# Autodesk Inventor assembly: 100-02
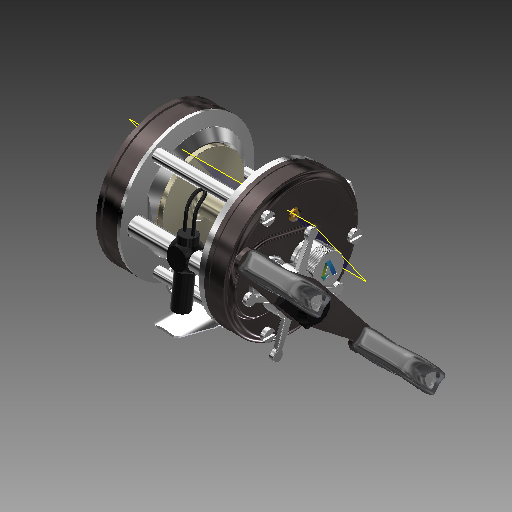
[picture p0: Inventor's stored thumbnail of the model, 512x512]
Saved by Autodesk Inventor 2019 (Build 230136000, 136)
## iProperties
Company: Autodesk Inc.
Created: 2017-06-27
Part Number: 100-02
Document SubType Name: Assembly
Designer: Autodesk Inc.
Mass: 263.654 g
Surface Area: 969.622 cm^2
Volume: 67.9846 cm^3
Density: 3.87815 g/cm^3
Author: Inventor
## Documents named in this file (31)
- C:\TEMP\Fishing Rod\Workspaces\_Fishing Reel Assembly.iam
- C:\TEMP\Fishing Rod\Workspaces\Reel Cage Assembly.iam
- C:\TEMP\Fishing Rod\Workspaces\Spool Assembly.iam
- C:\TEMP\Fishing Rod\Workspaces\Winding Assembly.iam
- C:\TEMP\Fishing Rod\Workspaces\Crankshaft Assembly.iam
- C:\TEMP\Fishing Rod\Workspaces\Crankshaft Spacer Tension Spring.ipt
- C:\TEMP\Fishing Rod\Workspaces\Handle Side Cover Assembly.iam
- C:\TEMP\Fishing Rod\Workspaces\Captive Cover Screw.ipt
- C:\TEMP\Fishing Rod\Workspaces\Plastic Bushing.ipt
- C:\TEMP\Fishing Rod\Workspaces\Front Drive Transfer Gear.iam
- C:\TEMP\Fishing Rod\Workspaces\Drag Adjustment Handle.ipt
- C:\TEMP\Fishing Rod\Workspaces\Plastic Crankshaft Spacer.ipt
- C:\TEMP\Fishing Rod\Workspaces\Spring Spacer.ipt
- C:\TEMP\Fishing Rod\Workspaces\Winding Handle.iam
- C:\TEMP\Fishing Rod\Workspaces\Crankshaft Cover.ipt
- C:\TEMP\Fishing Rod\Workspaces\Line Guide Tail Busing.ipt
- C:\TEMP\Fishing Rod\Workspaces\Line Guide Drive Shaft.ipt
- C:\TEMP\Fishing Rod\Workspaces\Follower Guide Pin Retainer.ipt
- C:\TEMP\Fishing Rod\Workspaces\Follower Guide Pin.ipt
- C:\TEMP\Fishing Rod\Workspaces\Line Guide.ipt
- C:\TEMP\Fishing Rod\Workspaces\Line Guide Shaft Housing.ipt
- C:\TEMP\Fishing Rod\Workspaces\Line Guide Head Bushing.ipt
- C:\TEMP\Fishing Rod\Workspaces\Locking Plate.ipt
- C:\TEMP\Fishing Rod\Workspaces\Winder Transfer Gear Spindle.ipt
- C:\TEMP\Fishing Rod\Workspaces\Winder Transfer Gear.iam
- C:\TEMP\Fishing Rod\Workspaces\Back Side Cover Assembly.iam
- C:\TEMP\Fishing Rod\Workspaces\Front Drive Transfer Gear\Design Accelerator\Bearing1.iam
- C:\TEMP\Fishing Rod\Workspaces\Main Bearing Cover.ipt
- C:\TEMP\Fishing Rod\Libraries\Content Center Files\en-US\ANSI B18.6.7M(03)\ANSI B18.6.7M - M2x0.4 x 6(3).ipt
- C:\TEMP\Fishing Rod\Libraries\Content Center Files\en-US\BS 4183(5)\BS 4183 - M3 x 5(2) I.ipt
- C:\TEMP\Fishing Rod\Workspaces\Back Drive Transfer Gear.iam
## Components (37 placed, 30 different names)
1. Reel Cage Assembly:1 [sub-assembly] — Mate:1, Insert:1, Mate:2, Angle:7, Insert:15, Mate:23, Mate:26, Mate:27, Mate:35, Mate:36, Tangent:6
2. Spool Assembly:1 [sub-assembly] — Mate:1, Mate:6, Mate:7, Tangent:2, Mate:8, Rotation:2, Rotation:3, Mate:20, Flush:1, Mate:27, Mate:34
3. Winding Assembly:1 [sub-assembly] — Insert:1, Mate:2, Insert:2, Insert:3, Mate:11
4. Crankshaft Assembly:1 [sub-assembly] — Insert:2, Mate:3, Angle:1, Mate:4, Angle:2, Mate:10, Angle:3, Angle:4, Rotation:1, Mate:29, Mate:30, Mate:37, Rotation:7
5. Crankshaft Spacer Tension Spring:1 — Mate:3, Angle:1, Mate:5
6. Crankshaft Spacer Tension Spring:2 — Mate:4, Angle:2, Mate:5, Tangent:3
7. Handle Side Cover Assembly:1 [sub-assembly] — Mate:6, Insert:3, Insert:4, Insert:6, Insert:22, Insert:23, Insert:36
8. Captive Cover Screw:1 — Insert:4
9. Captive Cover Screw:2 — Insert:36
10. Captive Cover Screw:3 — Insert:6
11. Plastic Bushing:1 — Insert:7
12. Front Drive Transfer Gear:1 [sub-assembly] — Mate:7, Tangent:2, Mate:8, Insert:7, Rotation:1, Rotation:2
13. Drag Adjustment Handle:1 — Insert:8, Tangent:4, Tangent:5, Rotation:7
14. Plastic Crankshaft Spacer:1 — Mate:10, Angle:3, Tangent:3, Insert:8
15. Spring Spacer:1 — Tangent:4, Tangent:5, Angle:4, Mate:11, Mate:28, Mate:37
16. Winding Handle:1 [sub-assembly] — Mate:28, Mate:29, Mate:30, Mate:31, Mate:32, Mate:33
17. Crankshaft Cover:1 — Insert:27, Mate:31, Mate:33
18. Line Guide Tail Busing:1 — Angle:7, Insert:12, Mate:17
19. Line Guide Drive Shaft:1 — Insert:12, Mate:15, Mate:19, Rotation:6
20. Follower Guide Pin Retainer:1 — Insert:14
21. Follower Guide Pin:1 — Insert:13
22. Line Guide:1 — Insert:13, Insert:14, Mate:18, Mate:34, Tangent:6
23. Line Guide Shaft Housing:1 — Mate:15, Mate:17, Mate:18, Angle:8, Mate:35, Mate:36
24. Line Guide Head Bushing:1 — Insert:28, Insert:35, Rotation:5, Rotation:6
25. Locking Plate:1 — Insert:15, Mate:19, Insert:28
26. Winder Transfer Gear:1 [sub-assembly] — Rotation:3, Mate:24, Rotation:4, Flush:1
27. Back Side Cover Assembly:1 [sub-assembly] — Mate:21, Mate:23, Insert:30, Mate:25, Insert:31, Mate:26, Insert:32, Insert:33, Insert:34
28. Winder Transfer Gear Spindle:1 — Insert:30, Mate:24
29. Bearing:1 [sub-assembly] — Mate:20, Mate:21, Mate:25
30. Main Bearing Cover:1 — Insert:31
31. Main Bearing Cover:2 — Insert:23
32. Bearing:2 [sub-assembly] — Insert:22
33. Slotted Pan Head Machine Screw - Metric M2x0.4 x 6:1 — Insert:34
34. Slotted Pan Head Machine Screw - Metric M2x0.4 x 6:2 — Insert:32
35. Slotted Pan Head Machine Screw - Metric M2x0.4 x 6:3 — Insert:33
36. BS 4183 Slotted Cheese Head Machine Screw - Metric M3 x 5:1 — Insert:27, Mate:32
37. Back Drive Transfer Gear:2 [sub-assembly] — Insert:35, Rotation:4, Rotation:5
## Relationships (72: Mate 31, Insert 22, RelateRotation 7, Angle 6, Tangent 5, Flush 1)
- Mate:1: Reel Cage Assembly:1 ↔ Spool Assembly:1
- Insert:1: Reel Cage Assembly:1 ↔ Winding Assembly:1
- Mate:2: Reel Cage Assembly:1 ↔ Winding Assembly:1
- Insert:2 (-1.5 mm): Winding Assembly:1 ↔ Crankshaft Assembly:1
- Mate:3: Crankshaft Assembly:1 ↔ Crankshaft Spacer Tension Spring:1
- Angle:1 (0 deg): Crankshaft Assembly:1 ↔ Crankshaft Spacer Tension Spring:1
- Mate:4: Crankshaft Assembly:1 ↔ Crankshaft Spacer Tension Spring:2
- Angle:2 (0 deg): Crankshaft Assembly:1 ↔ Crankshaft Spacer Tension Spring:2
- Mate:5 (1.4 mm): Crankshaft Spacer Tension Spring:1 ↔ Crankshaft Spacer Tension Spring:2
- Mate:6: Spool Assembly:1 ↔ Handle Side Cover Assembly:1
- Insert:3: Winding Assembly:1 ↔ Handle Side Cover Assembly:1
- Insert:4: Handle Side Cover Assembly:1 ↔ Captive Cover Screw:1
- Insert:6: Handle Side Cover Assembly:1 ↔ Captive Cover Screw:3
- Mate:7: Spool Assembly:1 ↔ Front Drive Transfer Gear:1
- Tangent:2: Spool Assembly:1 ↔ Front Drive Transfer Gear:1
- Mate:8: Spool Assembly:1 ↔ Front Drive Transfer Gear:1
- Insert:7: Plastic Bushing:1 ↔ Front Drive Transfer Gear:1
- Mate:10: Crankshaft Assembly:1 ↔ Plastic Crankshaft Spacer:1
- Angle:3 (0 deg): Crankshaft Assembly:1 ↔ Plastic Crankshaft Spacer:1
- Tangent:3: Crankshaft Spacer Tension Spring:2 ↔ Plastic Crankshaft Spacer:1
- Insert:8: Drag Adjustment Handle:1 ↔ Plastic Crankshaft Spacer:1
- Tangent:4: Drag Adjustment Handle:1 ↔ Spring Spacer:1
- Tangent:5: Drag Adjustment Handle:1 ↔ Spring Spacer:1
- Angle:4 (0 deg): Crankshaft Assembly:1 ↔ Spring Spacer:1
- Mate:11: Winding Assembly:1 ↔ Spring Spacer:1
- Angle:7 (90 deg): Reel Cage Assembly:1 ↔ Line Guide Tail Busing:1
- Insert:12: Line Guide Tail Busing:1 ↔ Line Guide Drive Shaft:1
- Insert:13: Follower Guide Pin:1 ↔ Line Guide:1
- Insert:14: Follower Guide Pin Retainer:1 ↔ Line Guide:1
- Mate:15: Line Guide Drive Shaft:1 ↔ Line Guide Shaft Housing:1
- Mate:17: Line Guide Tail Busing:1 ↔ Line Guide Shaft Housing:1
- Mate:18: Line Guide:1 ↔ Line Guide Shaft Housing:1
- Insert:15: Reel Cage Assembly:1 ↔ Locking Plate:1
- Mate:19: Line Guide Drive Shaft:1 ↔ Locking Plate:1
- Insert:22: Handle Side Cover Assembly:1 ↔ Bearing:2
- Insert:23: Handle Side Cover Assembly:1 ↔ Main Bearing Cover:2
- Insert:27: Crankshaft Cover:1 ↔ BS 4183 Slotted Cheese Head Machine Screw - Metric M3 x 5:1
- Insert:28: Line Guide Head Bushing:1 ↔ Locking Plate:1
- Rotation:1 [RelateRotation] (3.4 ul): Crankshaft Assembly:1 ↔ Front Drive Transfer Gear:1
- Rotation:2 [RelateRotation] (1 ul): Spool Assembly:1 ↔ Front Drive Transfer Gear:1
- Rotation:3 [RelateRotation] (0.2549 ul): Spool Assembly:1 ↔ Winder Transfer Gear:1
- Mate:20: Spool Assembly:1 ↔ Bearing:1
- Mate:21: Back Side Cover Assembly:1 ↔ Bearing:1
- Mate:23: Reel Cage Assembly:1 ↔ Back Side Cover Assembly:1
- Insert:30: Back Side Cover Assembly:1 ↔ Winder Transfer Gear Spindle:1
- Mate:24: Winder Transfer Gear:1 ↔ Winder Transfer Gear Spindle:1
- Mate:25: Back Side Cover Assembly:1 ↔ Bearing:1
- Insert:31 (1 mm): Back Side Cover Assembly:1 ↔ Main Bearing Cover:1
- Mate:26: Reel Cage Assembly:1 ↔ Back Side Cover Assembly:1
- Insert:32: Back Side Cover Assembly:1 ↔ Slotted Pan Head Machine Screw - Metric M2x0.4 x 6:2
- Insert:33: Back Side Cover Assembly:1 ↔ Slotted Pan Head Machine Screw - Metric M2x0.4 x 6:3
- Insert:34: Back Side Cover Assembly:1 ↔ Slotted Pan Head Machine Screw - Metric M2x0.4 x 6:1
- Insert:35: Line Guide Head Bushing:1 ↔ Back Drive Transfer Gear:2
- Rotation:4 [RelateRotation] (1.125 ul): Winder Transfer Gear:1 ↔ Back Drive Transfer Gear:2
- Flush:1: Spool Assembly:1 ↔ Winder Transfer Gear:1
- Mate:27 (0.25 mm): Reel Cage Assembly:1 ↔ Spool Assembly:1
- Rotation:5 [RelateRotation] (1 ul): Line Guide Head Bushing:1 ↔ Back Drive Transfer Gear:2
- Rotation:6 [RelateRotation] (1 ul): Line Guide Drive Shaft:1 ↔ Line Guide Head Bushing:1
- Mate:28: Spring Spacer:1 ↔ Winding Handle:1
- Mate:29: Crankshaft Assembly:1 ↔ Winding Handle:1
- Mate:30: Crankshaft Assembly:1 ↔ Winding Handle:1
- Mate:31: Winding Handle:1 ↔ Crankshaft Cover:1
- Mate:32: Winding Handle:1 ↔ BS 4183 Slotted Cheese Head Machine Screw - Metric M3 x 5:1
- Mate:33 (0.5 mm): Winding Handle:1 ↔ Crankshaft Cover:1
- Mate:34 (37 mm): Spool Assembly:1 ↔ Line Guide:1
- Angle:8 (180 deg): Line Guide Shaft Housing:1
- Mate:35: Reel Cage Assembly:1 ↔ Line Guide Shaft Housing:1
- Mate:36: Reel Cage Assembly:1 ↔ Line Guide Shaft Housing:1
- Insert:36: Handle Side Cover Assembly:1 ↔ Captive Cover Screw:2
- Mate:37: Crankshaft Assembly:1 ↔ Spring Spacer:1
- Tangent:6: Reel Cage Assembly:1 ↔ Line Guide:1
- Rotation:7 [RelateRotation] (1 ul): Crankshaft Assembly:1 ↔ Drag Adjustment Handle:1
